# Autodesk Inventor assembly: Assembly1
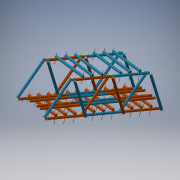
[picture p0: Inventor's stored thumbnail of the model, 180x180]
Saved by Autodesk Inventor 2016 (Build 200138000, 138)
## iProperties
Created: 2017-04-27
Part Number: Assembly1
Document SubType Name: Assembly
Designer: wtse3759
Author: wtse3759
## Documents named in this file (9)
- G:\Bridge\Assembly1.iam
- G:\Bridge\Straw.ipt
- G:\Bridge\toothpick2.ipt
- G:\Bridge\Straw open both sides.ipt
- G:\Bridge\Straw open one side with holes perp.ipt
- G:\Bridge\Straw middle.ipt
- G:\Bridge\Straw middle2.ipt
- G:\Bridge\Straw middle 3.ipt
- G:\Bridge\cap.ipt
## Components (134 placed, 8 different names)
1. toothpick2:3 — Mate:29, Mate:30, Mate:43, Mate:44
2. toothpick2:8 — Mate:23, Mate:26, Mate:42, Mate:482
3. toothpick2:10 — Mate:150, Mate:443
4. toothpick2:11 — Mate:11, Mate:31, Mate:149, Mate:442
5. toothpick2:12 — Mate:9, Mate:10, Mate:28, Mate:148
6. toothpick2:13 — Mate:8, Mate:25, Mate:484
7. Straw open both sides:1 — Mate:8, Mate:9, Insert:2, Tangent:5, Mate:48, Mate:49, Mate:50, Tangent:60, Angle:87, Angle:88, Insert:72
8. Straw open both sides:2 — Mate:10, Insert:2, Mate:11, Tangent:7, Mate:51, Mate:52, Mate:53, Tangent:61, Angle:91, Angle:92, Tangent:122, Tangent:123, Angle:95, Tangent:126, Insert:69
9. Straw:8 — Mate:23, Angle:52, Mate:148, Tangent:60
10. Straw:9 — Mate:25, Mate:26, Tangent:5
11. Straw:10 — Mate:28, Mate:30, Tangent:7, Tangent:15
12. Straw:11 — Mate:29, Angle:53, Mate:149, Tangent:61
13. Straw:12 — Mate:150, Angle:114, Tangent:159
14. Straw:14 — Mate:31, Mate:34, Tangent:16
15. toothpick2:14 — Mate:34, Mate:45, Mate:486
16. toothpick2:15 — Mate:303, Mate:383
17. toothpick2:16 — Mate:50, Mate:341
18. toothpick2:18 — Mate:48, Mate:336
19. toothpick2:19 — Mate:52, Mate:348
20. toothpick2:20 — Mate:49, Mate:338
21. toothpick2:21 — Mate:51, Mate:346
22. toothpick2:22 — Mate:53, Mate:354
23. Straw open both sides:4 — Mate:42, Mate:43, Tangent:15, Insert:6, Mate:57, Mate:58, Mate:59, Angle:52, Insert:70
24. Straw open both sides:5 — Mate:44, Mate:45, Insert:6, Tangent:16, Mate:60, Mate:61, Mate:62, Angle:53, Insert:74
25. toothpick2:23 — Mate:366
26. toothpick2:24 — Mate:357
27. toothpick2:25 — Mate:356
28. toothpick2:26 — Mate:57, Mate:373
29. toothpick2:27 — Mate:58, Mate:374
30. toothpick2:28 — Mate:59, Mate:375
31. toothpick2:29 — Mate:62, Mate:378
32. toothpick2:30 — Mate:61, Mate:377
33. toothpick2:31 — Mate:60, Mate:376
34. toothpick2:45 — Mate:307, Mate:385
35. toothpick2:46 — Mate:308, Mate:386
36. toothpick2:56 — Mate:309, Mate:387
37. toothpick2:63 — Mate:304, Mate:384
38. toothpick2:65 — Mate:302, Mate:382
39. toothpick2:70 — Mate:277, Mate:335
40. toothpick2:71 — Mate:278
41. toothpick2:72 — Mate:285, Mate:358
42. toothpick2:77 — Mate:279
43. toothpick2:78 — Mate:283, Mate:350
44. toothpick2:79 — Mate:284, Mate:351
45. toothpick2:80 — Mate:288, Mate:363
46. toothpick2:81 — Mate:289, Mate:360
47. toothpick2:82 — Mate:290, Mate:361
48. toothpick2:84 — Mate:281, Mate:282, Mate:311, Mate:314
49. toothpick2:85 — Mate:280, Mate:310, Mate:485
50. Straw open both sides:6 — Mate:277, Mate:278, Mate:279, Mate:280, Mate:281, Insert:65, Angle:73, Angle:74, Tangent:102, Tangent:103, Angle:75, Angle:85, Tangent:116, Tangent:118, Tangent:120, Insert:73
51. Straw open both sides:7 — Mate:282, Mate:283, Mate:284, Mate:285, Insert:65, Mate:286, Insert:66, Angle:76
52. toothpick2:86 — Mate:305, Mate:306
53. toothpick2:87 — Mate:291, Mate:317
54. toothpick2:88 — Mate:286, Mate:287, Mate:315, Mate:316
55. toothpick2:89 — Mate:301, Mate:312, Mate:313, Mate:483
56. Straw open one side with holes perp:5 — Mate:287, Insert:66, Mate:288, Mate:289, Mate:290, Mate:291, Angle:77, Angle:78, Angle:100
57. Straw:15 — Mate:310, Angle:73, Mate:312, Tangent:103
58. Straw:16 — Mate:311, Angle:74, Tangent:102, Mate:313
59. Straw:17 — Mate:314, Angle:75, Tangent:104
60. Straw open one side with holes perp:6 — Mate:306, Insert:68, Mate:307, Mate:308, Mate:309, Mate:318, Tangent:106, Tangent:107, Tangent:140, Tangent:141, Tangent:142
61. Straw open both sides:9 — Mate:301, Mate:302, Mate:303, Mate:304, Mate:305, Insert:68, Tangent:104, Tangent:105, Tangent:137, Tangent:138, Tangent:139, Insert:71
62. Straw:20 — Mate:315, Angle:76, Tangent:105
63. Straw:21 — Mate:317, Angle:78, Tangent:107
64. Straw:23 — Mate:316, Angle:77, Tangent:106
65. toothpick2:99 — Mate:318
66. Straw middle:10 — Mate:335, Angle:85, Mate:336, Tangent:116, Mate:410, Mate:412, Mate:414, Mate:415, Tangent:166, Tangent:167, Tangent:168
67. Straw middle:11 — Mate:338, Angle:87, Tangent:118
68. Straw middle:13 — Mate:346, Angle:91, Mate:350, Tangent:122, Mate:478, Mate:479, Tangent:169, Tangent:171
69. Straw middle:15 — Mate:348, Angle:92, Mate:351, Tangent:123, Mate:457, Mate:458, Angle:119, Angle:120, Angle:121, Tangent:170, Angle:122, Tangent:172
70. Straw middle:17 — Mate:341, Angle:88, Tangent:120, Mate:418, Mate:419, Mate:420, Mate:421, Angle:107, Angle:108, Angle:109, Angle:110, Tangent:165
71. Straw middle:19 — Mate:354, Angle:95, Mate:358, Tangent:126, Mate:426, Mate:428, Mate:430, Mate:446
72. Straw middle:21 — Mate:356, Mate:360, Tangent:153, Angle:123, Angle:124, Angle:125, Angle:126, Tangent:173, Tangent:174, Tangent:175, Tangent:176
73. Straw middle:22 — Mate:357, Mate:361, Mate:434, Tangent:155, Mate:451, Mate:453, Mate:454
74. Straw middle:24 — Mate:363, Angle:100, Mate:366, Tangent:151
75. Straw middle2:3 — Mate:373, Mate:382, Tangent:137
76. Straw middle2:5 — Mate:374, Mate:383, Tangent:138
77. Straw middle2:6 — Mate:376, Mate:385, Tangent:140
78. Straw middle2:7 — Mate:377, Mate:386, Tangent:141
79. Straw middle2:9 — Mate:375, Mate:384, Tangent:139
80. Straw middle2:10 — Mate:378, Mate:387, Tangent:142
81. toothpick2:112 — Mate:410
82. toothpick2:113 — Mate:419, Mate:424
83. toothpick2:114 — Mate:414
84. toothpick2:116 — Mate:418, Mate:425
85. toothpick2:117 — Mate:415
86. toothpick2:118 — Mate:412
87. Straw middle 3:6 — Mate:422, Angle:107, Mate:466, Tangent:165
88. Straw middle 3:7 — Mate:423, Angle:108, Mate:467, Tangent:168
89. toothpick2:119 — Mate:420, Mate:423
90. toothpick2:120 — Mate:421, Mate:422
91. Straw middle 3:8 — Mate:455, Mate:462, Mate:476, Angle:125, Tangent:174
92. Straw middle 3:9 — Mate:452, Mate:460, Mate:465, Angle:124, Tangent:175
93. Straw middle 3:10 — Mate:425, Angle:109, Mate:469, Tangent:166
94. Straw middle 3:12 — Mate:456, Mate:463, Mate:477, Angle:126, Tangent:173
95. Straw middle 3:13 — Mate:424, Angle:110, Mate:468, Tangent:167
96. toothpick2:121 — Mate:457, Mate:459
97. toothpick2:122 — Mate:458
98. toothpick2:123 — Mate:446
99. toothpick2:124 — Mate:461
100. toothpick2:125 — Mate:460
101. toothpick2:126 — Mate:463
102. toothpick2:127 — Mate:426, Mate:444
103. toothpick2:128 — Mate:464
104. toothpick2:129 — Mate:428, Mate:445
105. toothpick2:130 — Mate:430
106. toothpick2:132 — Mate:465
107. toothpick2:133 — Mate:454, Mate:456
108. toothpick2:134 — Mate:434, Mate:450
109. toothpick2:135 — Mate:462
110. toothpick2:138 — Mate:451, Mate:452
111. toothpick2:139 — Mate:453, Mate:455
112. Straw middle 3:14 — Mate:444, Mate:470, Mate:475, Angle:121, Tangent:169
113. Straw middle 3:15 — Mate:445, Mate:471, Mate:474, Angle:120, Tangent:170
114. Straw middle 3:16 — Mate:450, Mate:461, Mate:464, Angle:123, Tangent:176
115. Straw open one side with holes perp:8 — Mate:442, Insert:69, Mate:443, Tangent:151, Tangent:153, Tangent:155, Angle:114, Tangent:159
116. Straw middle 3:18 — Mate:459, Angle:119, Tangent:171
117. toothpick2:140 — Mate:467
118. toothpick2:141 — Mate:470
119. toothpick2:142 — Mate:468
120. toothpick2:143 — Mate:466
121. toothpick2:144 — Mate:471
122. toothpick2:146 — Mate:474
123. toothpick2:147 — Mate:469
124. toothpick2:148 — Mate:477
125. toothpick2:149 — Mate:476
126. toothpick2:150 — Mate:475
127. toothpick2:152 — Mate:479
128. toothpick2:153 — Mate:478, Mate:481
129. Straw middle 3:19 — Mate:481, Angle:122, Tangent:172
130. cap:1 — Mate:483, Insert:71
131. cap:2 — Mate:482, Insert:70
132. cap:3 — Mate:484, Insert:72
133. cap:4 — Mate:485, Insert:73
134. cap:5 — Mate:486, Insert:74
## Relationships (226: Mate 147, Tangent 40, Angle 28, Insert 11)
- Mate:8: toothpick2:13 ↔ Straw open both sides:1
- Mate:9: toothpick2:12 ↔ Straw open both sides:1
- Mate:10: toothpick2:12 ↔ Straw open both sides:2
- Insert:2: Straw open both sides:1 ↔ Straw open both sides:2
- Mate:11: toothpick2:11 ↔ Straw open both sides:2
- Mate:23: toothpick2:8 ↔ Straw:8
- Mate:25: toothpick2:13 ↔ Straw:9
- Mate:26: toothpick2:8 ↔ Straw:9
- Tangent:5: Straw open both sides:1 ↔ Straw:9
- Mate:28: toothpick2:12 ↔ Straw:10
- Mate:29: toothpick2:3 ↔ Straw:11
- Mate:30: toothpick2:3 ↔ Straw:10
- Tangent:7: Straw open both sides:2 ↔ Straw:10
- Mate:31: toothpick2:11 ↔ Straw:14
- Mate:34: Straw:14 ↔ toothpick2:14
- Mate:42: toothpick2:8 ↔ Straw open both sides:4
- Mate:43: toothpick2:3 ↔ Straw open both sides:4
- Tangent:15: Straw:10 ↔ Straw open both sides:4
- Mate:44: toothpick2:3 ↔ Straw open both sides:5
- Mate:45: toothpick2:14 ↔ Straw open both sides:5
- Insert:6: Straw open both sides:4 ↔ Straw open both sides:5
- Tangent:16: Straw:14 ↔ Straw open both sides:5
- Mate:48: Straw open both sides:1 ↔ toothpick2:18
- Mate:49: Straw open both sides:1 ↔ toothpick2:20
- Mate:50: Straw open both sides:1 ↔ toothpick2:16
- Mate:51: Straw open both sides:2 ↔ toothpick2:21
- Mate:52: Straw open both sides:2 ↔ toothpick2:19
- Mate:53: Straw open both sides:2 ↔ toothpick2:22
- Mate:57: Straw open both sides:4 ↔ toothpick2:26
- Mate:58: Straw open both sides:4 ↔ toothpick2:27
- Mate:59: Straw open both sides:4 ↔ toothpick2:28
- Mate:60: Straw open both sides:5 ↔ toothpick2:31
- Mate:61: Straw open both sides:5 ↔ toothpick2:30
- Mate:62: Straw open both sides:5 ↔ toothpick2:29
- Angle:52 (60 deg): Straw:8 ↔ Straw open both sides:4
- Mate:148: toothpick2:12 ↔ Straw:8
- Tangent:60: Straw open both sides:1 ↔ Straw:8
- Angle:53 (60 deg): Straw:11 ↔ Straw open both sides:5
- Mate:149: toothpick2:11 ↔ Straw:11
- Tangent:61: Straw open both sides:2 ↔ Straw:11
- Mate:150: toothpick2:10 ↔ Straw:12
- Mate:277: toothpick2:70 ↔ Straw open both sides:6
- Mate:278: toothpick2:71 ↔ Straw open both sides:6
- Mate:279: toothpick2:77 ↔ Straw open both sides:6
- Mate:280: toothpick2:85 ↔ Straw open both sides:6
- Mate:281: toothpick2:84 ↔ Straw open both sides:6
- Mate:282: toothpick2:84 ↔ Straw open both sides:7
- Mate:283: toothpick2:78 ↔ Straw open both sides:7
- Mate:284: toothpick2:79 ↔ Straw open both sides:7
- Mate:285: toothpick2:72 ↔ Straw open both sides:7
- Insert:65: Straw open both sides:6 ↔ Straw open both sides:7
- Mate:286: Straw open both sides:7 ↔ toothpick2:88
- Mate:287: toothpick2:88 ↔ Straw open one side with holes perp:5
- Insert:66: Straw open both sides:7 ↔ Straw open one side with holes perp:5
- Mate:288: toothpick2:80 ↔ Straw open one side with holes perp:5
- Mate:289: toothpick2:81 ↔ Straw open one side with holes perp:5
- Mate:290: toothpick2:82 ↔ Straw open one side with holes perp:5
- Mate:291: toothpick2:87 ↔ Straw open one side with holes perp:5
- Mate:301: toothpick2:89 ↔ Straw open both sides:9
- Mate:302: toothpick2:65 ↔ Straw open both sides:9
- Mate:303: toothpick2:15 ↔ Straw open both sides:9
- Mate:304: toothpick2:63 ↔ Straw open both sides:9
- Mate:305: toothpick2:86 ↔ Straw open both sides:9
- Mate:306: toothpick2:86 ↔ Straw open one side with holes perp:6
- Insert:68: Straw open one side with holes perp:6 ↔ Straw open both sides:9
- Mate:307: toothpick2:45 ↔ Straw open one side with holes perp:6
- Mate:308: toothpick2:46 ↔ Straw open one side with holes perp:6
- Mate:309: toothpick2:56 ↔ Straw open one side with holes perp:6
- Mate:310: toothpick2:85 ↔ Straw:15
- Angle:73 (120 deg): Straw open both sides:6 ↔ Straw:15
- Mate:311: toothpick2:84 ↔ Straw:16
- Angle:74 (60 deg): Straw open both sides:6 ↔ Straw:16
- Mate:312: toothpick2:89 ↔ Straw:15
- Tangent:102: Straw open both sides:6 ↔ Straw:16
- Tangent:103: Straw open both sides:6 ↔ Straw:15
- Mate:313: toothpick2:89 ↔ Straw:16
- Mate:314: toothpick2:84 ↔ Straw:17
- Angle:75 (300 deg): Straw open both sides:6 ↔ Straw:17
- Mate:315: toothpick2:88 ↔ Straw:20
- Angle:76 (240 deg): Straw open both sides:7 ↔ Straw:20
- Mate:316: toothpick2:88 ↔ Straw:23
- Angle:77 (120 deg): Straw open one side with holes perp:5 ↔ Straw:23
- Mate:317: toothpick2:87 ↔ Straw:21
- Angle:78 (60 deg): Straw open one side with holes perp:5 ↔ Straw:21
- Mate:318: Straw open one side with holes perp:6 ↔ toothpick2:99
- Tangent:104: Straw:17 ↔ Straw open both sides:9
- Tangent:105: Straw open both sides:9 ↔ Straw:20
- Tangent:106: Straw open one side with holes perp:6 ↔ Straw:23
- Tangent:107: Straw open one side with holes perp:6 ↔ Straw:21
- Mate:335: toothpick2:70 ↔ Straw middle:10
- Angle:85 (270 deg): Straw open both sides:6 ↔ Straw middle:10
- Mate:336: toothpick2:18 ↔ Straw middle:10
- Tangent:116: Straw open both sides:6 ↔ Straw middle:10
- Mate:338: toothpick2:20 ↔ Straw middle:11
- Mate:341: toothpick2:16 ↔ Straw middle:17
- Angle:87 (90 deg): Straw open both sides:1 ↔ Straw middle:11
- Angle:88 (90 deg): Straw open both sides:1 ↔ Straw middle:17
- Tangent:118: Straw open both sides:6 ↔ Straw middle:11
- Tangent:120: Straw open both sides:6 ↔ Straw middle:17
- Mate:346: toothpick2:21 ↔ Straw middle:13
- Mate:348: toothpick2:19 ↔ Straw middle:15
- Angle:91 (90 deg): Straw open both sides:2 ↔ Straw middle:13
- Angle:92 (90 deg): Straw open both sides:2 ↔ Straw middle:15
- Mate:350: toothpick2:78 ↔ Straw middle:13
- Mate:351: toothpick2:79 ↔ Straw middle:15
- Tangent:122: Straw open both sides:2 ↔ Straw middle:13
- Tangent:123: Straw open both sides:2 ↔ Straw middle:15
- Mate:354: toothpick2:22 ↔ Straw middle:19
- Mate:356: toothpick2:25 ↔ Straw middle:21
- Mate:357: toothpick2:24 ↔ Straw middle:22
- Angle:95 (90 deg): Straw open both sides:2 ↔ Straw middle:19
- Mate:358: toothpick2:72 ↔ Straw middle:19
- Mate:360: toothpick2:81 ↔ Straw middle:21
- Mate:361: toothpick2:82 ↔ Straw middle:22
- Tangent:126: Straw open both sides:2 ↔ Straw middle:19
- Mate:363: toothpick2:80 ↔ Straw middle:24
- Angle:100 (270 deg): Straw open one side with holes perp:5 ↔ Straw middle:24
- Mate:366: toothpick2:23 ↔ Straw middle:24
- Mate:373: toothpick2:26 ↔ Straw middle2:3
- Mate:374: toothpick2:27 ↔ Straw middle2:5
- Mate:375: toothpick2:28 ↔ Straw middle2:9
- Mate:376: toothpick2:31 ↔ Straw middle2:6
- Mate:377: toothpick2:30 ↔ Straw middle2:7
- Mate:378: toothpick2:29 ↔ Straw middle2:10
- Mate:382: toothpick2:65 ↔ Straw middle2:3
- Mate:383: toothpick2:15 ↔ Straw middle2:5
- Mate:384: toothpick2:63 ↔ Straw middle2:9
- Mate:385: toothpick2:45 ↔ Straw middle2:6
- Mate:386: toothpick2:46 ↔ Straw middle2:7
- Mate:387: toothpick2:56 ↔ Straw middle2:10
- Tangent:137: Straw open both sides:9 ↔ Straw middle2:3
- Tangent:138: Straw open both sides:9 ↔ Straw middle2:5
- Tangent:139: Straw open both sides:9 ↔ Straw middle2:9
- Tangent:140: Straw open one side with holes perp:6 ↔ Straw middle2:6
- Tangent:141: Straw open one side with holes perp:6 ↔ Straw middle2:7
- Tangent:142: Straw open one side with holes perp:6 ↔ Straw middle2:10
- Mate:410: Straw middle:10 ↔ toothpick2:112
- Mate:412: Straw middle:10 ↔ toothpick2:118
- Mate:414: Straw middle:10 ↔ toothpick2:114
- Mate:415: Straw middle:10 ↔ toothpick2:117
- Mate:418: Straw middle:17 ↔ toothpick2:116
- Mate:419: Straw middle:17 ↔ toothpick2:113
- Mate:420: Straw middle:17 ↔ toothpick2:119
- Mate:421: Straw middle:17 ↔ toothpick2:120
- Mate:422: Straw middle 3:6 ↔ toothpick2:120
- Angle:107 (270 deg): Straw middle:17 ↔ Straw middle 3:6
- Mate:423: Straw middle 3:7 ↔ toothpick2:119
- Angle:108 (270 deg): Straw middle:17 ↔ Straw middle 3:7
- Mate:424: toothpick2:113 ↔ Straw middle 3:13
- Mate:425: toothpick2:116 ↔ Straw middle 3:10
- Angle:109 (270 deg): Straw middle:17 ↔ Straw middle 3:10
- Angle:110 (270 deg): Straw middle:17 ↔ Straw middle 3:13
- Mate:426: Straw middle:19 ↔ toothpick2:127
- Mate:428: Straw middle:19 ↔ toothpick2:129
- Mate:430: Straw middle:19 ↔ toothpick2:130
- Mate:434: Straw middle:22 ↔ toothpick2:134
- Mate:442: toothpick2:11 ↔ Straw open one side with holes perp:8
- Insert:69: Straw open both sides:2 ↔ Straw open one side with holes perp:8
- Mate:443: toothpick2:10 ↔ Straw open one side with holes perp:8
- Tangent:151: Straw middle:24 ↔ Straw open one side with holes perp:8
- Tangent:153: Straw middle:21 ↔ Straw open one side with holes perp:8
- Tangent:155: Straw middle:22 ↔ Straw open one side with holes perp:8
- Mate:444: toothpick2:127 ↔ Straw middle 3:14
- Mate:445: toothpick2:129 ↔ Straw middle 3:15
- Mate:446: Straw middle:19 ↔ toothpick2:123
- Angle:114 (240 deg): Straw:12 ↔ Straw open one side with holes perp:8
- Tangent:159: Straw:12 ↔ Straw open one side with holes perp:8
- Mate:450: toothpick2:134 ↔ Straw middle 3:16
- Mate:451: Straw middle:22 ↔ toothpick2:138
- Mate:452: Straw middle 3:9 ↔ toothpick2:138
- Mate:453: Straw middle:22 ↔ toothpick2:139
- Mate:454: Straw middle:22 ↔ toothpick2:133
- Mate:455: Straw middle 3:8 ↔ toothpick2:139
- Mate:456: Straw middle 3:12 ↔ toothpick2:133
- Mate:457: Straw middle:15 ↔ toothpick2:121
- Mate:458: Straw middle:15 ↔ toothpick2:122
- Mate:459: toothpick2:121 ↔ Straw middle 3:18
- Angle:119 (90 deg): Straw middle:15 ↔ Straw middle 3:18
- Mate:460: Straw middle 3:9 ↔ toothpick2:125
- Mate:461: toothpick2:124 ↔ Straw middle 3:16
- Mate:462: Straw middle 3:8 ↔ toothpick2:135
- Mate:463: Straw middle 3:12 ↔ toothpick2:126
- Mate:464: toothpick2:128 ↔ Straw middle 3:16
- Mate:465: Straw middle 3:9 ↔ toothpick2:132
- Mate:466: Straw middle 3:6 ↔ toothpick2:143
- Mate:467: Straw middle 3:7 ↔ toothpick2:140
- Mate:468: Straw middle 3:13 ↔ toothpick2:142
- Mate:469: Straw middle 3:10 ↔ toothpick2:147
- Mate:470: Straw middle 3:14 ↔ toothpick2:141
- Mate:471: Straw middle 3:15 ↔ toothpick2:144
- Mate:474: Straw middle 3:15 ↔ toothpick2:146
- Mate:475: Straw middle 3:14 ↔ toothpick2:150
- Mate:476: Straw middle 3:8 ↔ toothpick2:149
- Mate:477: Straw middle 3:12 ↔ toothpick2:148
- Mate:478: Straw middle:13 ↔ toothpick2:153
- Mate:479: Straw middle:13 ↔ toothpick2:152
- Mate:481: toothpick2:153 ↔ Straw middle 3:19
- Mate:482: toothpick2:8 ↔ cap:2
- Insert:70: Straw open both sides:4 ↔ cap:2
- Mate:483: toothpick2:89 ↔ cap:1
- Insert:71: Straw open both sides:9 ↔ cap:1
- Mate:484: toothpick2:13 ↔ cap:3
- Insert:72: Straw open both sides:1 ↔ cap:3
- Mate:485: toothpick2:85 ↔ cap:4
- Insert:73: Straw open both sides:6 ↔ cap:4
- Mate:486: toothpick2:14 ↔ cap:5
- Insert:74: Straw open both sides:5 ↔ cap:5
- Tangent:165: Straw middle:17 ↔ Straw middle 3:6
- Tangent:166: Straw middle:10 ↔ Straw middle 3:10
- Tangent:167: Straw middle:10 ↔ Straw middle 3:13
- Tangent:168: Straw middle:10 ↔ Straw middle 3:7
- Angle:120 (270 deg): Straw middle:15 ↔ Straw middle 3:15
- Angle:121 (270 deg): Straw middle:15 ↔ Straw middle 3:14
- Tangent:169: Straw middle:13 ↔ Straw middle 3:14
- Tangent:170: Straw middle:15 ↔ Straw middle 3:15
- Tangent:171: Straw middle:13 ↔ Straw middle 3:18
- Angle:122 (270 deg): Straw middle:15 ↔ Straw middle 3:19
- Tangent:172: Straw middle:15 ↔ Straw middle 3:19
- Angle:123 (270 deg): Straw middle:21 ↔ Straw middle 3:16
- Angle:124 (270 deg): Straw middle:21 ↔ Straw middle 3:9
- Angle:125 (270 deg): Straw middle:21 ↔ Straw middle 3:8
- Angle:126 (270 deg): Straw middle:21 ↔ Straw middle 3:12
- Tangent:173: Straw middle:21 ↔ Straw middle 3:12
- Tangent:174: Straw middle:21 ↔ Straw middle 3:8
- Tangent:175: Straw middle:21 ↔ Straw middle 3:9
- Tangent:176: Straw middle:21 ↔ Straw middle 3:16
